# Autodesk Inventor assembly: ASSEMBLY DC MOTOR
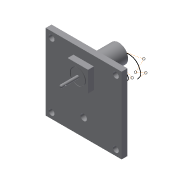
[picture p0: Inventor's stored thumbnail of the model, 180x180]
Saved by Autodesk Inventor 2019 (Build 230136000, 136)
## iProperties
Created: 2019-10-08
Part Number: ASSEMBLY DC MOTOR
Document SubType Name: Assembly
Designer: Admin
Author: Admin
## Documents named in this file (4)
- C:\Users\Admin\Documents\ASSEMBLY DC MOTOR.iam
- C:\Users\Admin\Documents\BOTTON.ipt
- C:\Users\Admin\Documents\dc motor.ipt
- C:\Users\Admin\Documents\dc motor nut.ipt
## Components (3 placed, 3 different names)
1. BOTTON:1 — Mate:1
2. dc motor:1 — Mate:1, Rotational:1
3. dc motor nut:1 — Rotational:1
## Relationships (2: Mate 1, RevoluteJoint 1)
- Mate:1: BOTTON:1 ↔ dc motor:1
- Rotational:1 [RevoluteJoint]: dc motor:1 ↔ dc motor nut:1
